# Autodesk Inventor assembly: holes_check_full
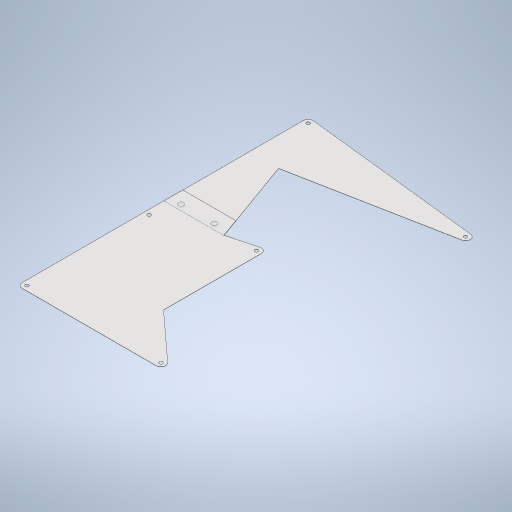
[picture p0: Inventor's stored thumbnail of the model, 512x512]
Saved by Autodesk Inventor 2024 (Build 280153000, 153)
## iProperties
Created: 2026-03-21
Part Number: holes_check_full
Document SubType Name: Assembly
Designer: schar
Author: schar
## Documents named in this file (3)
- C:\Users\schar\Desktop\tenSwitcHP\models\holes_check_full.iam
- C:\Users\schar\Desktop\tenSwitcHP\models\base_main_pcb_p1.ipt
- C:\Users\schar\Desktop\tenSwitcHP\models\base_main_pcb_p2.ipt
## Components (2 placed, 2 different names)
1. base_main_pcb_p1:1 — Mate:1, Mate:2, Mate:3
2. base_main_pcb_p2:1 — Mate:1, Mate:2, Mate:3
## Relationships (3: Mate 3)
- Mate:1: base_main_pcb_p1:1 ↔ base_main_pcb_p2:1
- Mate:2: base_main_pcb_p1:1 ↔ base_main_pcb_p2:1
- Mate:3: base_main_pcb_p1:1 ↔ base_main_pcb_p2:1
